# Autodesk Inventor assembly: mountAssembly
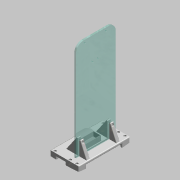
[picture p0: Inventor's stored thumbnail of the model, 180x180]
Saved by Autodesk Inventor 2020 (Build 240168000, 168)
## iProperties
Part Number: mountAssembly
Document SubType Name: Assembly
Designer: Watchdog
Author: Watchdog
## Documents named in this file (4)
- C:\Users\Watchdog\OneDrive - Flinders\ENGR0001\3_Design\mountAssembly.iam
- C:\Users\Watchdog\OneDrive - Flinders\ENGR0001\3_Design\2_plate\mountPlate.ipt
- C:\Users\Watchdog\OneDrive - Flinders\ENGR0001\3_Design\2_base\under.ipt
- C:\Users\Watchdog\OneDrive - Flinders\ENGR0001\3_Design\container.ipt
## Components (3 placed, 3 different names)
1. mountPlate:1 — Mate:3, Mate:7, Mate:8
2. under:1 — Mate:1, Flush:1, Mate:2, Mate:3, Mate:4, Mate:5, Mate:6, Mate:7, Mate:8
3. container:1 — Mate:4, Mate:5, Mate:6
## Relationships (9: Mate 8, Flush 1)
- Mate:1: under:1
- Flush:1: under:1
- Mate:2: under:1
- Mate:3: mountPlate:1 ↔ under:1
- Mate:4: under:1 ↔ container:1
- Mate:5 (1.5 mm): under:1 ↔ container:1
- Mate:6 (1.5 mm): under:1 ↔ container:1
- Mate:7: mountPlate:1 ↔ under:1
- Mate:8: mountPlate:1 ↔ under:1
